# Autodesk Inventor assembly: Задний_столб_MIR1
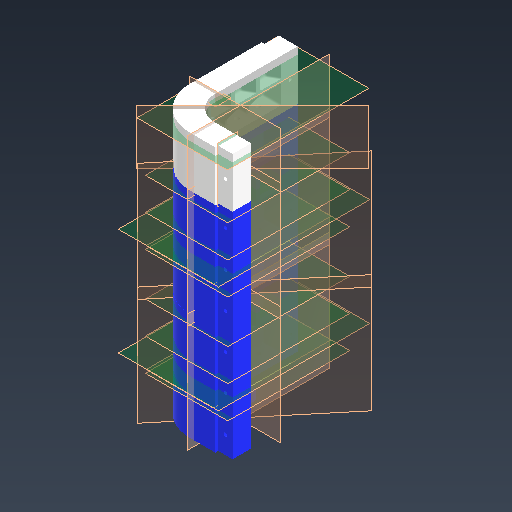
[picture p0: Inventor's stored thumbnail of the model, 512x512]
Saved by Autodesk Inventor 2023.2 (Build 272271030, 271C)
## iProperties
Created: 2025-09-30
Part Number: Задний_столб_MIR1
Document SubType Name: Assembly
Designer: Олег Коноваленко
Author: Олег Коноваленко
## Documents named in this file (4)
- D:\!Rover\Rover\Rover_construction\Задний_столб_MIR1.iam
- D:\!Rover\Rover\Rover_construction\Столб_версия_2.0_MIR3.ipt
- D:\!Rover\Rover\Rover_construction\Столб_версия_2.0_MIR4.ipt
- D:\!Rover\Rover\Rover_construction\Верхняя часть столба зада_MIR1.ipt
## Components (3 placed, 3 different names)
1. Столб_версия_2.0_MIR3:1 — Заподлицо:2, Заподлицо:1, Совмещение:1
2. Столб_версия_2.0_MIR4:1 — Заподлицо:2, Заподлицо:1, Совмещение:1, Заподлицо:4, Заподлицо:3, Совмещение:2
3. Верхняя часть столба зада_MIR1:1 — Заподлицо:4, Заподлицо:3, Совмещение:2
## Relationships (6: Flush 4, Mate 2)
- Заподлицо:2 [Flush]: Столб_версия_2.0_MIR3:1 ↔ Столб_версия_2.0_MIR4:1
- Заподлицо:1 [Flush]: Столб_версия_2.0_MIR3:1 ↔ Столб_версия_2.0_MIR4:1
- Совмещение:1 [Mate]: Столб_версия_2.0_MIR3:1 ↔ Столб_версия_2.0_MIR4:1
- Заподлицо:4 [Flush]: Столб_версия_2.0_MIR4:1 ↔ Верхняя часть столба зада_MIR1:1
- Заподлицо:3 [Flush]: Столб_версия_2.0_MIR4:1 ↔ Верхняя часть столба зада_MIR1:1
- Совмещение:2 [Mate]: Столб_версия_2.0_MIR4:1 ↔ Верхняя часть столба зада_MIR1:1
